# Autodesk Inventor assembly: s-assy-gripper
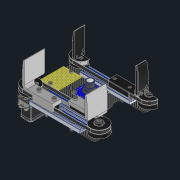
[picture p0: Inventor's stored thumbnail of the model, 180x180]
Saved by Autodesk Inventor 2022 (Build 260153000, 153)
## iProperties
Created: 2021-08-06
Part Number: s-assy-gripper
Document SubType Name: Assembly
Designer: yuta0
Mass: 588.108 g
Surface Area: 2137.5 cm^2
Volume: 253.038 cm^3
Density: 2.32419 g/cm^3
Author: yuta0
## Documents named in this file (27)
- C:\Users\yuta0\Documents\GitHub\catchrobo_hardware\assy-robot\s-assy-gripper.iam
- C:\Users\yuta0\Documents\GitHub\catchrobo_hardware\assy-robot\carbon_plate14.ipt
- C:\Users\yuta0\Documents\GitHub\catchrobo_hardware\assy-robot\mrs20-100.ipt
- C:\Users\yuta0\Documents\GitHub\catchrobo_hardware\assy-robot\mr-20cs_1.iam
- C:\Users\yuta0\Documents\GitHub\catchrobo_hardware\assy-robot\belt4.ipt
- C:\Users\yuta0\Documents\GitHub\catchrobo_hardware\assy-robot\base37.ipt
- C:\Users\yuta0\Documents\GitHub\catchrobo_hardware\assy-robot\USB Cam model ELP-USBFHD01M-L21.ipt
- C:\Users\yuta0\Documents\GitHub\catchrobo_hardware\assy-robot\CB3-5.ipt
- C:\Users\yuta0\Documents\GitHub\catchrobo_hardware\assy-robot\base38.ipt
- C:\Users\yuta0\Documents\GitHub\catchrobo_hardware\assy-robot\CB3-30.ipt
- C:\Users\yuta0\Documents\GitHub\catchrobo_hardware\assy-robot\LBNR4.ipt
- C:\Users\yuta0\Documents\GitHub\catchrobo_hardware\assy-robot\ARU-2010.ipt
- C:\Users\yuta0\Documents\GitHub\catchrobo_hardware\assy-robot\CB2-4.ipt
- C:\Users\yuta0\Documents\GitHub\catchrobo_hardware\assy-robot\d_type_board.ipt
- C:\Users\yuta0\Documents\GitHub\catchrobo_hardware\assy-robot\hexagonal_spacer_M3_5mm.ipt
- C:\Users\yuta0\Documents\GitHub\catchrobo_hardware\assy-robot\LBNR3.ipt
- C:\Users\yuta0\Documents\GitHub\catchrobo_hardware\assy-robot\steel_plate1.ipt
- C:\Users\yuta0\Documents\GitHub\catchrobo_hardware\assy-robot\CBSTNR3-16.ipt
- C:\Users\yuta0\Documents\GitHub\catchrobo_hardware\assy-robot\s-assy-rc_servo.iam
- C:\Users\yuta0\Documents\GitHub\catchrobo_hardware\assy-robot\s-assy-gripper_tentioner.iam
- C:\Users\yuta0\Documents\GitHub\catchrobo_hardware\assy-robot\FU650AD5-C6.ipt
- C:\Users\yuta0\Documents\GitHub\catchrobo_hardware\assy-robot\base21.ipt
- C:\Users\yuta0\Documents\GitHub\catchrobo_hardware\assy-robot\CBSTSR4-14.ipt
- C:\Users\yuta0\Documents\GitHub\catchrobo_hardware\assy-robot\base22.ipt
- C:\Users\yuta0\Documents\GitHub\catchrobo_hardware\assy-robot\CB3-10.ipt
- C:\Users\yuta0\Documents\GitHub\catchrobo_hardware\assy-robot\base49.ipt
- C:\Users\yuta0\Documents\GitHub\catchrobo_hardware\assy-robot\CB4-20.ipt
## Components (85 placed, 26 different names)
1. carbon_plate14:1 — メイト:1, メイト:2, メイト:3, メイト:51, メイト:52, メイト:53, メイト:88, メイト:89, メイト:90, メイト:92, 角度:1, メイト:98, メイト:102, メイト:103, メイト:104, メイト:105, メイト:106, メイト:107, メイト:109, メイト:110, メイト:111, メイト:113, メイト:139, メイト:140, メイト:141, メイト:142, メイト:143, メイト:144, メイト:147, メイト:150, メイト:183, メイト:197, メイト:200, 角度:4, 角度:5, メイト:201, メイト:202, メイト:203, メイト:207, メイト:208
2. s-assy-rc_servo:1 [sub-assembly] — メイト:139, メイト:140, メイト:141, メイト:145, メイト:146
3. s-assy-rc_servo:2 [sub-assembly] — メイト:142, メイト:143, メイト:144, メイト:153, メイト:154
4. s-assy-gripper_tentioner:1 [sub-assembly] — メイト:147, メイト:149
5. USB Cam model ELP-USBFHD01M-L21:1 — メイト:51, メイト:52, メイト:53, メイト:99, メイト:100, メイト:101
6. hexagonal_spacer_M3_5mm:1 — メイト:106, メイト:107, メイト:108, メイト:114
7. LBNR3:1 — メイト:108, メイト:109
8. LBNR3:2 — メイト:112, メイト:113
9. hexagonal_spacer_M3_5mm:2 — メイト:110, メイト:111, メイト:112
10. d_type_board:1 — メイト:104, メイト:105, メイト:114, メイト:115, メイト:116, メイト:117, メイト:118
11. CB3-5:11 — メイト:115, メイト:116
12. CB3-5:12 — メイト:117, メイト:118
13. belt4:1 — メイト:145, メイト:146, メイト:149
14. belt4:2 — メイト:152, メイト:153, メイト:154, メイト:234
15. FU650AD5-C6:1 — メイト:197, メイト:198, 角度:5
16. FU650AD5-C6:2 — メイト:199, メイト:200, 角度:4
17. base21:1 — メイト:201, メイト:202, メイト:203, メイト:204, メイト:205
18. base21:2 — メイト:206, メイト:207, メイト:208, メイト:209, メイト:210
19. s-assy-gripper_tentioner:2 [sub-assembly] — メイト:150, メイト:152
20. CB3-30:1 — メイト:88, メイト:89
21. CB3-30:2
22. CB3-30:3
23. CB3-30:4
24. CB3-30:5
25. CB3-30:6
26. ARU-2010:1 — メイト:98, メイト:99
27. CB2-4:1 — メイト:100, メイト:101
28. CB2-4:2 — メイト:102, メイト:103
29. ARU-2010:2
30. CB2-4:3
31. CB2-4:6
32. ARU-2010:3
33. CB2-4:4
34. CB2-4:7
35. ARU-2010:4
36. CB2-4:5
37. CB2-4:8
38. steel_plate1:1 — メイト:129, メイト:130, メイト:131, メイト:133, メイト:134, メイト:135, メイト:219, メイト:220, メイト:221
39. CBSTNR3-16:1 — メイト:132, メイト:133
40. CBSTNR3-16:2 — メイト:134, メイト:135
41. base37:1 — メイト:45, メイト:46, メイト:47, メイト:70, メイト:71, メイト:72
42. base38:1 — メイト:70, メイト:71, メイト:72, メイト:129, メイト:130, メイト:131, メイト:132
43. mr-20cs_1:1 [sub-assembly] — メイト:7, メイト:8, フラッシュ:1, メイト:45, メイト:46, メイト:47
44. mrs20-100:1 — フラッシュ:1, メイト:1, メイト:2, メイト:3, メイト:7, メイト:8, メイト:199
45. CBSTSR4-14:3
46. LBNR4:1 — メイト:90, 角度:2, メイト:210
47. CBSTSR4-14:4 — メイト:206
48. LBNR4:2 — メイト:92, 角度:1, 角度:2, メイト:209
49. CB3-10:4 — メイト:223
50. CB3-10:3 — メイト:222
51. base22:2 — メイト:219, メイト:220, メイト:221, メイト:222, メイト:223
52. steel_plate1:4
53. CBSTNR3-16:7
54. CBSTNR3-16:8
55. base37:4
56. base38:4
57. mr-20cs_1:4 [sub-assembly]
58. mrs20-100:4
59. CBSTSR4-14:7
60. LBNR4:7
61. CBSTSR4-14:8
62. LBNR4:8
63. CB3-10:7
64. CB3-10:8
65. base22:4
66. CB4-20:2 — メイト:237, メイト:238, メイト:239
67. CB4-20:1 — メイト:235, メイト:236
68. base49:1 — メイト:227, メイト:234, 正接:1, メイト:236, メイト:239
69. base37:2 — メイト:226, メイト:227, 正接:1, メイト:235, メイト:237
70. mr-20cs_1:2 [sub-assembly] — メイト:226, メイト:238
71. mrs20-100:2 — メイト:183, メイト:198
72. CBSTSR4-14:2
73. LBNR4:3 — メイト:205
74. LBNR4:4 — メイト:204
75. CBSTSR4-14:1
76. CB4-20:3
77. CB4-20:4
78. base49:2
79. base37:5
80. mr-20cs_1:5 [sub-assembly]
81. mrs20-100:5
82. CBSTSR4-14:9
83. LBNR4:9
84. LBNR4:10
85. CBSTSR4-14:10
## Component patterns: (6 elements, first: CB3-30:1), (4 elements, first: ARU-2010:1 + CB2-4:1 + CB2-4:2), (2 elements, first: steel_plate1:1 + CBSTNR3-16:1 + CBSTNR3-16:2 + base37:1 + base38:1 + mr-20cs_1:1 + mrs20-100:1 + CBSTSR4-14:3 + LBNR4:1 + CBSTSR4-14:4 + LBNR4:2 + CB3-10:4 + CB3-10:3 + base22:2), (2 elements, first: CB4-20:2 + CB4-20:1 + base49:1 + base37:2 + mr-20cs_1:2 + mrs20-100:2 + CBSTSR4-14:2 + LBNR4:3 + LBNR4:4 + CBSTSR4-14:1)
## Relationships (113: Mate 105, Angle 5, Flush 2, Tangent 1)
- フラッシュ:1 [Flush]: mr-20cs_1:1 ↔ mrs20-100:1
- [Flush]: mr-20cs_1:2 ↔ mrs20-100:2
- メイト:1 [Mate]: carbon_plate14:1 ↔ mrs20-100:1
- メイト:2 [Mate]: carbon_plate14:1 ↔ mrs20-100:1
- メイト:3 [Mate]: carbon_plate14:1 ↔ mrs20-100:1
- メイト:7 [Mate] (0.1 mm): mr-20cs_1:1 ↔ mrs20-100:1
- メイト:8 [Mate] (0.15 mm): mr-20cs_1:1 ↔ mrs20-100:1
- メイト:45 [Mate]: base37:1 ↔ mr-20cs_1:1
- メイト:46 [Mate]: base37:1 ↔ mr-20cs_1:1
- メイト:47 [Mate]: base37:1 ↔ mr-20cs_1:1
- メイト:51 [Mate] (10 mm): carbon_plate14:1 ↔ USB Cam model ELP-USBFHD01M-L21:1
- メイト:52 [Mate]: carbon_plate14:1 ↔ USB Cam model ELP-USBFHD01M-L21:1
- メイト:53 [Mate]: carbon_plate14:1 ↔ USB Cam model ELP-USBFHD01M-L21:1
- メイト:70 [Mate]: base37:1 ↔ base38:1
- メイト:71 [Mate]: base37:1 ↔ base38:1
- メイト:72 [Mate]: base37:1 ↔ base38:1
- メイト:88 [Mate]: carbon_plate14:1 ↔ CB3-30:1
- メイト:89 [Mate]: carbon_plate14:1 ↔ CB3-30:1
- メイト:90 [Mate]: carbon_plate14:1 ↔ LBNR4:1
- メイト:92 [Mate]: carbon_plate14:1 ↔ LBNR4:2
- 角度:1 [Angle] (0 deg): carbon_plate14:1 ↔ LBNR4:2
- 角度:2 [Angle] (0 deg): LBNR4:1 ↔ LBNR4:2
- メイト:98 [Mate]: carbon_plate14:1 ↔ ARU-2010:1
- メイト:99 [Mate]: USB Cam model ELP-USBFHD01M-L21:1 ↔ ARU-2010:1
- メイト:100 [Mate]: USB Cam model ELP-USBFHD01M-L21:1 ↔ CB2-4:1
- メイト:101 [Mate]: USB Cam model ELP-USBFHD01M-L21:1 ↔ CB2-4:1
- メイト:102 [Mate]: carbon_plate14:1 ↔ CB2-4:2
- メイト:103 [Mate]: carbon_plate14:1 ↔ CB2-4:2
- メイト:104 [Mate]: carbon_plate14:1 ↔ d_type_board:1
- メイト:105 [Mate]: carbon_plate14:1 ↔ d_type_board:1
- メイト:106 [Mate]: carbon_plate14:1 ↔ hexagonal_spacer_M3_5mm:1
- メイト:107 [Mate]: carbon_plate14:1 ↔ hexagonal_spacer_M3_5mm:1
- メイト:108 [Mate]: hexagonal_spacer_M3_5mm:1 ↔ LBNR3:1
- メイト:109 [Mate]: carbon_plate14:1 ↔ LBNR3:1
- メイト:110 [Mate]: carbon_plate14:1 ↔ hexagonal_spacer_M3_5mm:2
- メイト:111 [Mate]: carbon_plate14:1 ↔ hexagonal_spacer_M3_5mm:2
- メイト:112 [Mate]: LBNR3:2 ↔ hexagonal_spacer_M3_5mm:2
- メイト:113 [Mate]: carbon_plate14:1 ↔ LBNR3:2
- メイト:114 [Mate]: hexagonal_spacer_M3_5mm:1 ↔ d_type_board:1
- メイト:115 [Mate]: d_type_board:1 ↔ CB3-5:11
- メイト:116 [Mate]: d_type_board:1 ↔ CB3-5:11
- メイト:117 [Mate]: d_type_board:1 ↔ CB3-5:12
- メイト:118 [Mate]: d_type_board:1 ↔ CB3-5:12
- [Mate]: mrs20-100:1 ↔ CBSTSR4-14:3
- [Mate]: mrs20-100:1 ↔ CBSTSR4-14:3
- [Mate]: mrs20-100:1 ↔ CBSTSR4-14:4
- [Mate]: mrs20-100:1 ↔ CBSTSR4-14:4
- メイト:129 [Mate]: steel_plate1:1 ↔ base38:1
- メイト:130 [Mate]: steel_plate1:1 ↔ base38:1
- メイト:131 [Mate]: steel_plate1:1 ↔ base38:1
- メイト:132 [Mate]: CBSTNR3-16:1 ↔ base38:1
- メイト:133 [Mate]: steel_plate1:1 ↔ CBSTNR3-16:1
- メイト:134 [Mate]: steel_plate1:1 ↔ CBSTNR3-16:2
- メイト:135 [Mate]: steel_plate1:1 ↔ CBSTNR3-16:2
- [Mate]: steel_plate1:1 ↔ CB3-10:4
- [Mate]: steel_plate1:1 ↔ CB3-10:3
- メイト:139 [Mate]: carbon_plate14:1 ↔ s-assy-rc_servo:1
- メイト:140 [Mate]: carbon_plate14:1 ↔ s-assy-rc_servo:1
- メイト:141 [Mate]: carbon_plate14:1 ↔ s-assy-rc_servo:1
- メイト:142 [Mate]: carbon_plate14:1 ↔ s-assy-rc_servo:2
- メイト:143 [Mate]: carbon_plate14:1 ↔ s-assy-rc_servo:2
- メイト:144 [Mate]: carbon_plate14:1 ↔ s-assy-rc_servo:2
- メイト:145 [Mate]: s-assy-rc_servo:1 ↔ belt4:1
- メイト:146 [Mate] (0.5 mm): s-assy-rc_servo:1 ↔ belt4:1
- メイト:147 [Mate]: carbon_plate14:1 ↔ s-assy-gripper_tentioner:1
- メイト:149 [Mate]: s-assy-gripper_tentioner:1 ↔ belt4:1
- メイト:150 [Mate]: carbon_plate14:1 ↔ s-assy-gripper_tentioner:2
- メイト:152 [Mate]: belt4:2 ↔ s-assy-gripper_tentioner:2
- メイト:153 [Mate]: s-assy-rc_servo:2 ↔ belt4:2
- メイト:154 [Mate] (0.5 mm): s-assy-rc_servo:2 ↔ belt4:2
- [Mate] (0.1 mm): mr-20cs_1:2 ↔ mrs20-100:2
- [Mate] (0.15 mm): mr-20cs_1:2 ↔ mrs20-100:2
- [Mate]: base37:2 ↔ mr-20cs_1:2
- [Angle] (0 deg): LBNR4:3 ↔ LBNR4:4
- [Mate]: mrs20-100:2 ↔ CBSTSR4-14:2
- [Mate]: mrs20-100:2 ↔ CBSTSR4-14:2
- [Mate]: mrs20-100:2 ↔ CBSTSR4-14:1
- [Mate]: mrs20-100:2 ↔ CBSTSR4-14:1
- [Mate]: carbon_plate14:1 ↔ CBSTSR4-14:2
- [Mate]: carbon_plate14:1 ↔ CBSTSR4-14:1
- メイト:183 [Mate]: carbon_plate14:1 ↔ mrs20-100:2
- [Mate]: LBNR4:4 ↔ CBSTSR4-14:1
- [Mate]: CBSTSR4-14:2 ↔ LBNR4:3
- メイト:197 [Mate]: carbon_plate14:1 ↔ FU650AD5-C6:1
- メイト:198 [Mate]: FU650AD5-C6:1 ↔ mrs20-100:2
- メイト:199 [Mate]: FU650AD5-C6:2 ↔ mrs20-100:1
- メイト:200 [Mate]: carbon_plate14:1 ↔ FU650AD5-C6:2
- 角度:4 [Angle] (0 deg): carbon_plate14:1 ↔ FU650AD5-C6:2
- 角度:5 [Angle] (0 deg): carbon_plate14:1 ↔ FU650AD5-C6:1
- メイト:201 [Mate]: carbon_plate14:1 ↔ base21:1
- メイト:202 [Mate]: carbon_plate14:1 ↔ base21:1
- メイト:203 [Mate]: carbon_plate14:1 ↔ base21:1
- メイト:204 [Mate]: base21:1 ↔ LBNR4:4
- メイト:205 [Mate]: base21:1 ↔ LBNR4:3
- メイト:206 [Mate]: base21:2 ↔ CBSTSR4-14:4
- メイト:207 [Mate]: carbon_plate14:1 ↔ base21:2
- メイト:208 [Mate]: carbon_plate14:1 ↔ base21:2
- メイト:209 [Mate]: base21:2 ↔ LBNR4:2
- メイト:210 [Mate]: base21:2 ↔ LBNR4:1
- メイト:219 [Mate]: steel_plate1:1 ↔ base22:2
- メイト:220 [Mate]: steel_plate1:1 ↔ base22:2
- メイト:221 [Mate]: steel_plate1:1 ↔ base22:2
- メイト:222 [Mate]: CB3-10:3 ↔ base22:2
- メイト:223 [Mate]: CB3-10:4 ↔ base22:2
- メイト:226 [Mate]: base37:2 ↔ mr-20cs_1:2
- メイト:227 [Mate]: base49:1 ↔ base37:2
- メイト:234 [Mate]: belt4:2 ↔ base49:1
- 正接:1 [Tangent]: base49:1 ↔ base37:2
- メイト:235 [Mate]: CB4-20:1 ↔ base37:2
- メイト:236 [Mate]: CB4-20:1 ↔ base49:1
- メイト:237 [Mate]: CB4-20:2 ↔ base37:2
- メイト:238 [Mate]: CB4-20:2 ↔ mr-20cs_1:2
- メイト:239 [Mate]: CB4-20:2 ↔ base49:1
## Named parameters: d280_d22 = 0.1 mm, d281_d23 = 0.15 mm, d282_d214 = 0 mm, d283_d215 = 0 mm, d284_d216 = 0 mm, d285_d217 = 0 mm, d286_d170 = 0 deg, d289_d106 = 0 mm, d297_d26 = 0 mm
